# Autodesk Inventor assembly: Shower head
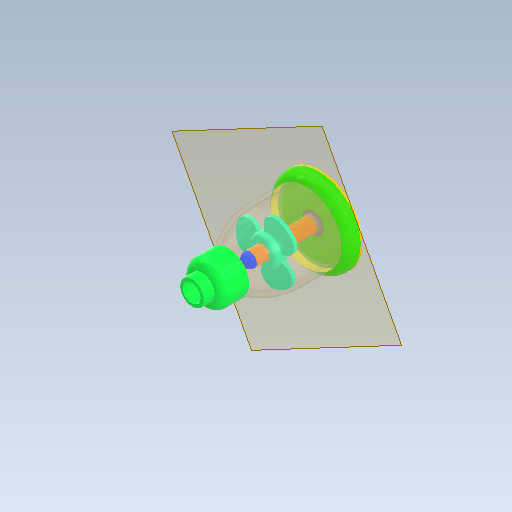
[picture p0: Inventor's stored thumbnail of the model, 512x512]
Saved by Autodesk Inventor 2021 (Build 250183000, 183)
## iProperties
Created: 2021-07-30
Part Number: Shower head
Document SubType Name: Assembly
Designer: Shammy Haider
Author: Shammy Haider
## Documents named in this file (5)
- D:\Designing\Autodesk inventor\Shower head\Shower head.iam
- D:\Designing\Autodesk inventor\Shower head\Bottum.ipt
- D:\Designing\Autodesk inventor\Shower head\fan.ipt
- D:\Designing\Autodesk inventor\Shower head\Outer.ipt
- D:\Designing\Autodesk inventor\Shower head\upper.ipt
## Components (4 placed, 4 different names)
1. Bottum:1 — Mate:1, Mate:2, Mate:3, Mate:4, Flush:1
2. fan:1 — Mate:5, Angle:1
3. Outer:1 — Mate:3, Mate:4, Mate:5, Mate:6, Mate:7
4. upper:1 — Mate:6, Mate:7
## Relationships (9: Mate 7, Flush 1, Angle 1)
- Mate:1: Bottum:1
- Mate:2: Bottum:1
- Mate:3: Bottum:1 ↔ Outer:1
- Mate:4: Bottum:1 ↔ Outer:1
- Mate:5: fan:1 ↔ Outer:1
- Mate:6: Outer:1 ↔ upper:1
- Mate:7 (-3 mm): Outer:1 ↔ upper:1
- Flush:1 (3.75 mm): Bottum:1
- Angle:1 (0 deg): fan:1
